# Autodesk Inventor assembly: Antriebsstrang
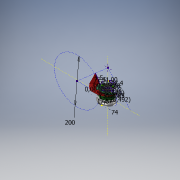
[picture p0: Inventor's stored thumbnail of the model, 180x180]
Saved by Autodesk Inventor 2018.3 (Build 223284000, 284)
## iProperties
Created: 2018-06-25
Part Number: Antriebsstrang
Material: Generisch
Document SubType Name: Assembly
Designer: JochenAlt
Author: JochenAlt
## Documents named in this file (16)
- D:\Projects\FlowerPot\CAD\DriveChain.iam
- D:\Projects\FlowerPot\CAD\OmniWheel.ipt
- D:\Projects\FlowerPot\CAD\Mounting Hub.ipt
- D:\Projects\FlowerPot\CAD\Avago Encoder.iam
- D:\Projects\FlowerPot\CAD\HarmonicDrive.ipt
- D:\Projects\FlowerPot\CAD\HarmonicDrive-Axis.ipt
- C:\Users\JochenAlt\Documents\Inventor\Content Center Files\R2018\de-DE\AS 1420\AS 1420 - 1973 - M3 x 8.ipt
- C:\Users\JochenAlt\Documents\Inventor\Content Center Files\R2018\de-DE\DIN 912\DIN 912 - M2 x 0,4 x 8 x 7.ipt
- C:\Users\JochenAlt\Documents\Inventor\Content Center Files\R2018\de-DE\DIN 934\DIN 934 - M2 x 0,4.ipt
- D:\Projects\FlowerPot\CAD\BushOmniWheel.ipt
- D:\Projects\FlowerPot\CAD\EncoderBushLeft.ipt
- D:\Projects\FlowerPot\CAD\EncoderBushRight.ipt
- C:\Users\JochenAlt\Documents\Inventor\Content Center Files\R2018\de-DE\DIN BEARING(1)\DIN 625 SKF - SKF 623.ipt
- D:\Projects\FlowerPot\CAD\Motor.iam
- D:\Projects\FlowerPot\CAD\PlanetaryGear\PlanetaryGear.iam
- D:\Projects\FlowerPot\CAD\BushingPlanetaryGearLeft.ipt
## Components (29 placed, 15 different names)
1. OmniWheel:1 — Passend:1, Passend:3, Passend:4, Passend:5, Passend:6, Passend:7, Passend:8, Passend:9, Passend:10, Passend:11, Passend:12, Passend:14, Passend:16, Passend:18, Passend:20, Passend:22, Passend:24, Fluchtend:1, Passend:55
2. Mounting Hub:1 — Passend:1, Passend:25, Passend:30, Passend:31, Passend:55
3. Avago Encoder:1 [sub-assembly] — Passend:34, Passend:37, Passend:46
4. HarmonicDrive3:1 — Passend:70, Passend:71, Passend:82
5. AS 1420 - Metrisch M3 x 8:1 — Passend:3, Passend:4
6. AS 1420 - Metrisch M3 x 8:2 — Passend:5, Passend:6, Passend:30
7. AS 1420 - Metrisch M3 x 8:3 — Passend:7, Passend:8
8. AS 1420 - Metrisch M3 x 8:4 — Passend:9, Passend:10
9. DIN 934 - ersetzt durch DIN EN 24032/28673/28674 M2:1 — Passend:13, Passend:14
10. DIN 934 - ersetzt durch DIN EN 24032/28673/28674 M2:2 — Passend:15, Passend:16
11. DIN 934 - ersetzt durch DIN EN 24032/28673/28674 M2:3 — Passend:17, Passend:18
12. DIN 934 - ersetzt durch DIN EN 24032/28673/28674 M2:4 — Passend:19, Passend:20
13. DIN 934 - ersetzt durch DIN EN 24032/28673/28674 M2:5 — Passend:21, Passend:22
14. DIN 934 - ersetzt durch DIN EN 24032/28673/28674 M2:6 — Passend:23, Passend:24
15. HarmonicDrive-Axis:2 — Passend:25, Fluchtend:1, Passend:29, Passend:34, Passend:35, Passend:38, Passend:67, Passend:72, Passend:77, Passend:78
16. BushOmniWheel:1 — Passend:29, Passend:31, Passend:73
17. EncoderBushLeft:1 — Passend:35, Passend:37, Passend:75
18. EncoderBushRight:1 — Passend:38, Passend:46, Passend:76
19. DIN 625 SKF SKF 623:1 — Passend:70, Passend:71, Passend:72, Passend:73, Passend:75
20. DIN 625 SKF SKF 623:2 — Passend:76, Passend:77, Passend:79
21. Motor:1 [sub-assembly] — Passend:66, Passend:68, Passend:69, Passend:81, Passend:82, Passend:83
22. PlanetaryGear:1 [sub-assembly] — Passend:67, Passend:68, Passend:69, Passend:80, Passend:81, Passend:83
23. BushingPlanetaryGearLeft:2 — Passend:78, Passend:79, Passend:80
24. DIN 912 - ersetzt durch DIN EN ISO 4762 M2 x 8:1 — Passend:11, Passend:12, Passend:13
25. DIN 912 - ersetzt durch DIN EN ISO 4762 M2 x 8:2 — Passend:23
26. DIN 912 - ersetzt durch DIN EN ISO 4762 M2 x 8:3 — Passend:21
27. DIN 912 - ersetzt durch DIN EN ISO 4762 M2 x 8:4 — Passend:19
28. DIN 912 - ersetzt durch DIN EN ISO 4762 M2 x 8:5 — Passend:17
29. DIN 912 - ersetzt durch DIN EN ISO 4762 M2 x 8:6 — Passend:15
## Component patterns: (6 elements, first: DIN 912 - ersetzt durch DIN EN ISO 4762 M2 x 8:1)
## Relationships (51: Mate 50, Flush 1)
- Passend:1 [Mate]: OmniWheel:1 ↔ Mounting Hub:1
- Passend:3 [Mate]: OmniWheel:1 ↔ AS 1420 - Metrisch M3 x 8:1
- Passend:4 [Mate]: OmniWheel:1 ↔ AS 1420 - Metrisch M3 x 8:1
- Passend:5 [Mate]: OmniWheel:1 ↔ AS 1420 - Metrisch M3 x 8:2
- Passend:6 [Mate]: OmniWheel:1 ↔ AS 1420 - Metrisch M3 x 8:2
- Passend:7 [Mate]: OmniWheel:1 ↔ AS 1420 - Metrisch M3 x 8:3
- Passend:8 [Mate]: OmniWheel:1 ↔ AS 1420 - Metrisch M3 x 8:3
- Passend:9 [Mate]: OmniWheel:1 ↔ AS 1420 - Metrisch M3 x 8:4
- Passend:10 [Mate]: OmniWheel:1 ↔ AS 1420 - Metrisch M3 x 8:4
- Passend:11 [Mate]: OmniWheel:1 ↔ DIN 912 - ersetzt durch DIN EN ISO 4762 M2 x 8:1
- Passend:12 [Mate]: OmniWheel:1 ↔ DIN 912 - ersetzt durch DIN EN ISO 4762 M2 x 8:1
- Passend:13 [Mate]: DIN 934 - ersetzt durch DIN EN 24032/28673/28674 M2:1 ↔ DIN 912 - ersetzt durch DIN EN ISO 4762 M2 x 8:1
- Passend:14 [Mate]: OmniWheel:1 ↔ DIN 934 - ersetzt durch DIN EN 24032/28673/28674 M2:1
- Passend:15 [Mate]: DIN 934 - ersetzt durch DIN EN 24032/28673/28674 M2:2 ↔ DIN 912 - ersetzt durch DIN EN ISO 4762 M2 x 8:6
- Passend:16 [Mate]: OmniWheel:1 ↔ DIN 934 - ersetzt durch DIN EN 24032/28673/28674 M2:2
- Passend:17 [Mate]: DIN 934 - ersetzt durch DIN EN 24032/28673/28674 M2:3 ↔ DIN 912 - ersetzt durch DIN EN ISO 4762 M2 x 8:5
- Passend:18 [Mate]: OmniWheel:1 ↔ DIN 934 - ersetzt durch DIN EN 24032/28673/28674 M2:3
- Passend:19 [Mate]: DIN 934 - ersetzt durch DIN EN 24032/28673/28674 M2:4 ↔ DIN 912 - ersetzt durch DIN EN ISO 4762 M2 x 8:4
- Passend:20 [Mate]: OmniWheel:1 ↔ DIN 934 - ersetzt durch DIN EN 24032/28673/28674 M2:4
- Passend:21 [Mate]: DIN 934 - ersetzt durch DIN EN 24032/28673/28674 M2:5 ↔ DIN 912 - ersetzt durch DIN EN ISO 4762 M2 x 8:3
- Passend:22 [Mate]: OmniWheel:1 ↔ DIN 934 - ersetzt durch DIN EN 24032/28673/28674 M2:5
- Passend:23 [Mate]: DIN 934 - ersetzt durch DIN EN 24032/28673/28674 M2:6 ↔ DIN 912 - ersetzt durch DIN EN ISO 4762 M2 x 8:2
- Passend:24 [Mate]: OmniWheel:1 ↔ DIN 934 - ersetzt durch DIN EN 24032/28673/28674 M2:6
- Passend:25 [Mate]: Mounting Hub:1 ↔ HarmonicDrive-Axis:2
- Fluchtend:1 [Flush]: OmniWheel:1 ↔ HarmonicDrive-Axis:2
- Passend:29 [Mate]: HarmonicDrive-Axis:2 ↔ BushOmniWheel:1
- Passend:30 [Mate]: Mounting Hub:1 ↔ AS 1420 - Metrisch M3 x 8:2
- Passend:31 [Mate]: Mounting Hub:1 ↔ BushOmniWheel:1
- Passend:34 [Mate]: Avago Encoder:1 ↔ HarmonicDrive-Axis:2
- Passend:35 [Mate]: HarmonicDrive-Axis:2 ↔ EncoderBushLeft:1
- Passend:37 [Mate] (-1 mm): Avago Encoder:1 ↔ EncoderBushLeft:1
- Passend:38 [Mate]: HarmonicDrive-Axis:2 ↔ EncoderBushRight:1
- Passend:46 [Mate] (-1.25 mm): Avago Encoder:1 ↔ EncoderBushRight:1
- Passend:55 [Mate]: OmniWheel:1 ↔ Mounting Hub:1
- Passend:66 [Mate]: Motor:1
- Passend:67 [Mate]: HarmonicDrive-Axis:2 ↔ PlanetaryGear:1
- Passend:68 [Mate]: Motor:1 ↔ PlanetaryGear:1
- Passend:69 [Mate]: Motor:1 ↔ PlanetaryGear:1
- Passend:70 [Mate]: HarmonicDrive3:1 ↔ DIN 625 SKF SKF 623:1
- Passend:71 [Mate]: HarmonicDrive3:1 ↔ DIN 625 SKF SKF 623:1
- Passend:72 [Mate]: HarmonicDrive-Axis:2 ↔ DIN 625 SKF SKF 623:1
- Passend:73 [Mate]: BushOmniWheel:1 ↔ DIN 625 SKF SKF 623:1
- Passend:75 [Mate]: EncoderBushLeft:1 ↔ DIN 625 SKF SKF 623:1
- Passend:76 [Mate]: EncoderBushRight:1 ↔ DIN 625 SKF SKF 623:2
- Passend:77 [Mate]: HarmonicDrive-Axis:2 ↔ DIN 625 SKF SKF 623:2
- Passend:78 [Mate]: HarmonicDrive-Axis:2 ↔ BushingPlanetaryGearLeft:2
- Passend:79 [Mate]: DIN 625 SKF SKF 623:2 ↔ BushingPlanetaryGearLeft:2
- Passend:80 [Mate]: PlanetaryGear:1 ↔ BushingPlanetaryGearLeft:2
- Passend:81 [Mate]: Motor:1 ↔ PlanetaryGear:1
- Passend:82 [Mate]: HarmonicDrive3:1 ↔ Motor:1
- Passend:83 [Mate]: Motor:1 ↔ PlanetaryGear:1
